# Autodesk Inventor assembly: fanasm
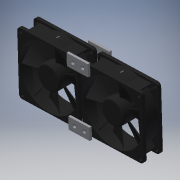
[picture p0: Inventor's stored thumbnail of the model, 180x180]
Saved by Autodesk Inventor 2017 (Build 210142000, 142)
## iProperties
Created: 2017-03-09
Part Number: fanasm
Document SubType Name: Assembly
Designer: LaFaucheuse
Author: LaFaucheuse
## Documents named in this file (3)
- D:\[DATA]\[SW]\projetLDB\fanasm.iam
- D:\[DATA]\[SW]\projetLDB\rapid_fan_grill_pattern_04.iam
- D:\[DATA]\[SW]\projetLDB\attache.ipt
## Components (6 placed, 2 different names)
1. rapid_fan_grill_pattern_04:1 [sub-assembly] — Placage:1, Placage:3, Placage:6, Placage:8, Placage:10, Placage:11, Placage:13, Placage:15
2. rapid_fan_grill_pattern_04:2 [sub-assembly] — Placage:2, Placage:4, Placage:5, Placage:7, Placage:9, Placage:12, Placage:14, Placage:16
3. attache:1 — Placage:5, Placage:6, Placage:7, Placage:8
4. attache:2 — Placage:13, Placage:14, Placage:15, Placage:16
5. attache:3 — Placage:9, Placage:10, Placage:11, Placage:12
6. attache:4 — Placage:1, Placage:2, Placage:3, Placage:4
## Relationships (16: Mate 16)
- Placage:1 [Mate]: rapid_fan_grill_pattern_04:1 ↔ attache:4
- Placage:2 [Mate]: rapid_fan_grill_pattern_04:2 ↔ attache:4
- Placage:3 [Mate]: rapid_fan_grill_pattern_04:1 ↔ attache:4
- Placage:4 [Mate]: rapid_fan_grill_pattern_04:2 ↔ attache:4
- Placage:5 [Mate]: rapid_fan_grill_pattern_04:2 ↔ attache:1
- Placage:6 [Mate]: rapid_fan_grill_pattern_04:1 ↔ attache:1
- Placage:7 [Mate]: rapid_fan_grill_pattern_04:2 ↔ attache:1
- Placage:8 [Mate]: rapid_fan_grill_pattern_04:1 ↔ attache:1
- Placage:9 [Mate]: rapid_fan_grill_pattern_04:2 ↔ attache:3
- Placage:10 [Mate]: rapid_fan_grill_pattern_04:1 ↔ attache:3
- Placage:11 [Mate]: rapid_fan_grill_pattern_04:1 ↔ attache:3
- Placage:12 [Mate]: rapid_fan_grill_pattern_04:2 ↔ attache:3
- Placage:13 [Mate]: rapid_fan_grill_pattern_04:1 ↔ attache:2
- Placage:14 [Mate]: rapid_fan_grill_pattern_04:2 ↔ attache:2
- Placage:15 [Mate]: rapid_fan_grill_pattern_04:1 ↔ attache:2
- Placage:16 [Mate]: rapid_fan_grill_pattern_04:2 ↔ attache:2
